# Autodesk Inventor assembly: mirrorHolder
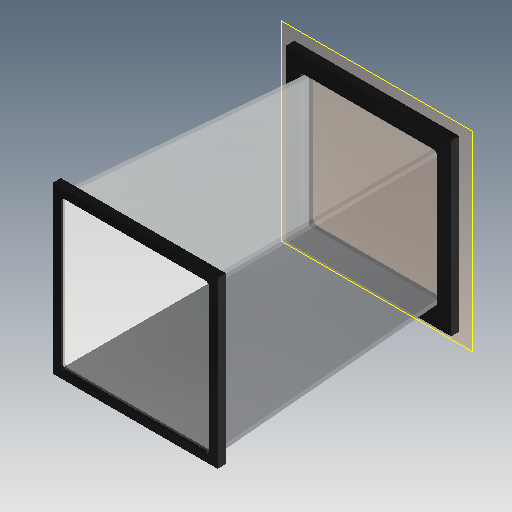
[picture p0: Inventor's stored thumbnail of the model, 512x512]
Saved by Autodesk Inventor 2018 (Build 220112000, 112)
## iProperties
Created: 2015-10-27
Part Number: mirrorHolder
Document SubType Name: Assembly
Designer: Sawaiz
Author: Sawaiz
## Documents named in this file (5)
- C:\Users\sawaiz\OneDrive\projects\modularRICH\mirror\mirrorHolder.iam
- C:\Users\sawaiz\OneDrive\projects\modularRICH\mirror\mirrorFrontFrame.ipt
- C:\Users\sawaiz\OneDrive\projects\modularRICH\mirror\mirrorSides.ipt
- C:\Users\sawaiz\OneDrive\projects\modularRICH\mirror\mirrorBackFrame.ipt
- C:\Users\sawaiz\OneDrive\projects\modularRICH\modularRICH.xlsx
## Components (6 placed, 3 different names)
1. mirrorFrontFrame:1 — Mate:1, Mate:2, Mate:3, Mate:4, Mate:5, Mate:6, Mate:7, Mate:8, Flush:1, Symmetry:1, Symmetry:2, Symmetry:3
2. mirrorSides:1 — Mate:1, Mate:8, Mate:9, Mate:11
3. mirrorSides:2 — Mate:4, Mate:5, Mate:11
4. mirrorSides:3 — Mate:2, Mate:7, Mate:9, Mate:10
5. mirrorSides:4 — Mate:3, Mate:6, Mate:10
6. mirrorBackFrame:1 — Flush:2, Symmetry:1, Symmetry:2, Symmetry:3
## Relationships (16: Mate 11, Symmetry 3, Flush 2)
- Mate:1: mirrorFrontFrame:1 ↔ mirrorSides:1
- Mate:2: mirrorFrontFrame:1 ↔ mirrorSides:3
- Mate:3: mirrorFrontFrame:1 ↔ mirrorSides:4
- Mate:4: mirrorFrontFrame:1 ↔ mirrorSides:2
- Mate:5: mirrorFrontFrame:1 ↔ mirrorSides:2
- Mate:6: mirrorFrontFrame:1 ↔ mirrorSides:4
- Mate:7: mirrorFrontFrame:1 ↔ mirrorSides:3
- Mate:8: mirrorFrontFrame:1 ↔ mirrorSides:1
- Mate:9: mirrorSides:1 ↔ mirrorSides:3
- Mate:10: mirrorSides:3 ↔ mirrorSides:4
- Mate:11: mirrorSides:1 ↔ mirrorSides:2
- Flush:1 (-185.8249 mm): mirrorFrontFrame:1
- Flush:2: mirrorBackFrame:1
- Symmetry:1: mirrorFrontFrame:1 ↔ mirrorBackFrame:1
- Symmetry:2: mirrorFrontFrame:1 ↔ mirrorBackFrame:1
- Symmetry:3: mirrorFrontFrame:1 ↔ mirrorBackFrame:1
## Named parameters: frameAcrylicThickness = 9.525 mm, internalAcrylicThickness = 6.35 mm, aerogelThickness = 30 mm, aerogelWidth = 110 mm, aerogelHeight = 110 mm, height = 127 mm, width = 127 mm, depth = 247.57228 mm, mirrorAngle = 2.5 deg, detectorWidth = 52 mm, detectorHeight = 52 mm, mirrorThickness = 3.175 mm, fresnelThickness = 0.254 mm, grooveDensity = 125, focalLength = 185.82488 mm, ior = 1.49, centerThickness = 1.27 mm, fresnelAngle = 90 deg, fresnelEffectiveDiameter = 152.4 mm, oRingWidth = 1.5875 mm, sensorHolderDepth = 19.05 mm, aerogelClearence = 3.175 mm, backplanePCBWidth = 76.2 mm, backplanePCBHeight = 76.2 mm, backplaneHoleOffsett = 6.35 mm, backplanePostionOffsett = 12.7 mm, moduleSlotClearence = 0.79375 mm, testMountHeight = 300 mm, testMountWidth = 300 mm, testMountLength = 500 mm, plasticThickness = 6.35 mm, aerogelHolderDepth = 38.24501 mm, caseThickness = 6.35 mm, alignmantGrooveDepth = 1.5875 mm, alignmentGrooveDepth = 1.5875 mm, alignmentGrooveClearance = 0.1016 mm, frontPanelThickness = 1.5875 mm, fresnelGrooveWidth = 9.525 mm, lensInsetDepth = 6.35 mm, lensMountThickness = 9.525 mm, lensDiameter = 101.6 mm, lensCenterThickness = 16.99999 mm
